# Autodesk Inventor assembly: 240614_사다리
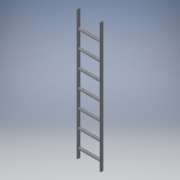
[picture p0: Inventor's stored thumbnail of the model, 180x180]
Saved by Autodesk Inventor 2016 (Build 200138000, 138)
## iProperties
Created: 2024-06-14
Part Number: 240614_사다리
Material: 일반
Document SubType Name: Assembly
Designer: pc
Author: pc
## Documents named in this file (3)
- D:\CAD_HCH\240614\240614_사다리.iam
- D:\CAD_HCH\240614\240614_day3060_500.ipt
- D:\CAD_HCH\240614\240614_day3060_3000.ipt
## Components (9 placed, 2 different names)
1. 240614_day3060_3000:1 — 메이트:1, 플러쉬:1, 플러쉬:3
2. 240614_day3060_3000:2 — 메이트:2, 플러쉬:2
3. 240614_day3060_500:1 — 메이트:1, 메이트:2, 플러쉬:1, 플러쉬:2, 플러쉬:3
4. 240614_day3060_500:10
5. 240614_day3060_500:11
6. 240614_day3060_500:12
7. 240614_day3060_500:13
8. 240614_day3060_500:14
9. 240614_day3060_500:15
## Component patterns: (7 elements, first: 240614_day3060_500:1)
## Relationships (5: Flush 3, Mate 2)
- 메이트:1 [Mate]: 240614_day3060_3000:1 ↔ 240614_day3060_500:1
- 메이트:2 [Mate]: 240614_day3060_3000:2 ↔ 240614_day3060_500:1
- 플러쉬:1 [Flush]: 240614_day3060_3000:1 ↔ 240614_day3060_500:1
- 플러쉬:2 [Flush]: 240614_day3060_3000:2 ↔ 240614_day3060_500:1
- 플러쉬:3 [Flush] (200 mm): 240614_day3060_3000:1 ↔ 240614_day3060_500:1
